# Autodesk Inventor assembly: Подставка под мотор
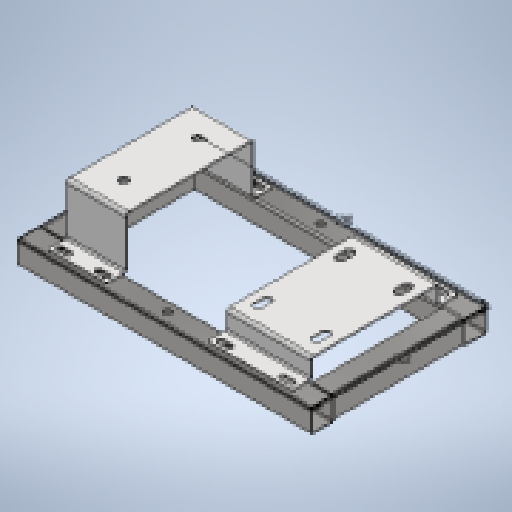
[picture p0: Inventor's stored thumbnail of the model, 512x512]
Saved by Autodesk Inventor 2026.2 (Build 302298010, 298A)
## iProperties
Created: 2026-06-04
Part Number: Подставка под мотор
Document SubType Name: Assembly
Designer: admin
_SolveAssemblyDoc: Frame Generator Solve Assembly
_Version: 25.0.0
Author: admin
## Documents named in this file (5)
- C:\Users\admin\Documents\Inventor\DMF-Disk-Micro-Filter\Подставка под мотор.iam
- C:\Users\admin\Documents\Inventor\DMF-Disk-Micro-Filter\скетч подставка.ipt
- C:\Users\admin\Documents\Inventor\DMF-Disk-Micro-Filter\Подставка под мотор\Frame\Frame 1780576945572.iam
- C:\Users\admin\Documents\Inventor\DMF-Disk-Micro-Filter\DMF Подставка ркдуктор.ipt
- C:\Users\admin\Documents\Inventor\DMF-Disk-Micro-Filter\DMF Подставка ркдуктор_CPY.ipt
## Components (4 placed, 4 different names)
1. скетч подставка:1
2. DMF Подставка подшипник:1 — Mate:1, Mate:4
3. DMF Подставка ркдуктор:1 — Mate:2, Flush:1, Mate:3
4. Frame 1780576945572:1 [sub-assembly] — Mate:1, Mate:2, Flush:1
## Relationships (5: Mate 4, Flush 1)
- Mate:1: DMF Подставка подшипник:1 ↔ Frame 1780576945572:1
- Mate:2: DMF Подставка ркдуктор:1 ↔ Frame 1780576945572:1
- Flush:1 (45 mm): DMF Подставка ркдуктор:1 ↔ Frame 1780576945572:1
- Mate:3: DMF Подставка ркдуктор:1
- Mate:4: DMF Подставка подшипник:1
